# Autodesk Inventor assembly: E1_Base_Meca_IIm_Ligne
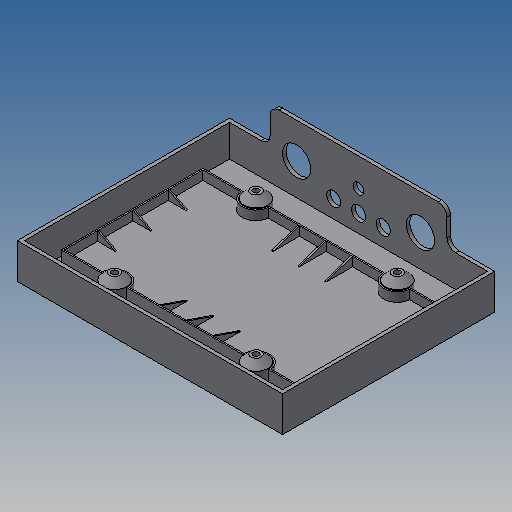
[picture p0: Inventor's stored thumbnail of the model, 512x512]
Saved by Autodesk Inventor 2025.3 (Build 293356000, 356)
## iProperties
Created: 2026-08-27
Part Number: E1_Base_Meca_IIm_Ligne
Project: Nom Projet
Description: Ens. Nom Ensemble
Document SubType Name: Assembly
Designer: jules
Mass: 0.0729356 g
Surface Area: 891.448 cm^2
Volume: 72.9356 cm^3
Density: 0.001 g/cm^3
Author: jules
## Documents named in this file (3)
- C:\Users\jules\OneDrive\PCB_Perso\PCB_IIm_Ligne\Meca_IIm_Ligne\E1_Base_Meca_IIm_Ligne.iam
- C:\Users\jules\OneDrive\PCB_Perso\PCB_IIm_Ligne\Meca_IIm_Ligne\Base_Meca_IIm_Ligne.ipt
- C:\Users\jules\OneDrive\PCB_Perso\PCB_IIm_Ligne\Meca_IIm_Ligne\Leste_Meca_IIm_Ligne.ipt
## Components (2 placed, 2 different names)
1. Base_Meca_IIm_Ligne:1 — Placage:1, Placage:2, Placage:3
2. Leste_Meca_IIm_Ligne:1 — Placage:1, Placage:2, Placage:3
## Relationships (3: Mate 3)
- Placage:1 [Mate]: Base_Meca_IIm_Ligne:1 ↔ Leste_Meca_IIm_Ligne:1
- Placage:2 [Mate]: Base_Meca_IIm_Ligne:1 ↔ Leste_Meca_IIm_Ligne:1
- Placage:3 [Mate]: Base_Meca_IIm_Ligne:1 ↔ Leste_Meca_IIm_Ligne:1
